# Autodesk Inventor assembly: 1000_Device
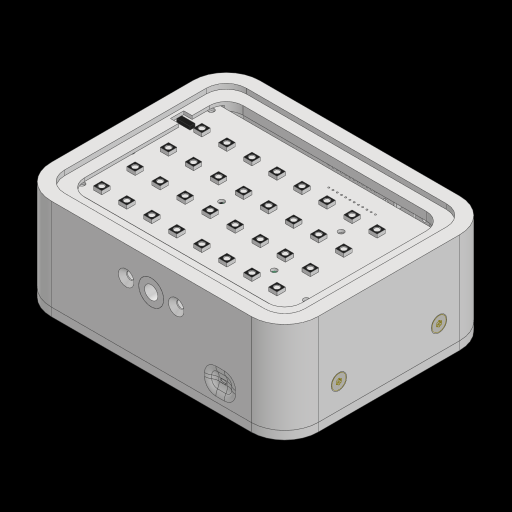
[picture p0: Inventor's stored thumbnail of the model, 512x512]
Saved by Autodesk Inventor 2024 (Build 280153000, 153)
## iProperties
Created: 2023-07-20
Part Number: 1000_Device
Document SubType Name: Assembly
Designer: Philipp
Author: Philipp
## Documents named in this file (10)
- C:\Users\phili\Documents\GitHub\PICO\20 Hardware\1000_Device.iam
- C:\Users\phili\Documents\GitHub\PICO\20 Hardware\020_Battery_4Cell.ipt
- C:\Users\phili\Documents\GitHub\PICO\20 Hardware\100_PICO_Mainboard.ipt
- C:\Users\phili\Documents\GitHub\PICO\20 Hardware\110_PICO_Daughterboard.ipt
- C:\Users\phili\Documents\GitHub\PICO\20 Hardware\SSD1306\Pantalla OLED 0.96'' 128x64.iam
- C:\Users\phili\Documents\GitHub\PICO\20 Hardware\210_Shell_External.ipt
- C:\Users\phili\Documents\GitHub\PICO\20 Hardware\220_Frame_Mainboard.ipt
- C:\Users\phili\Documents\GitHub\PICO\20 Hardware\250_CameraMount.ipt
- C:\Users\phili\Documents\GitHub\PICO\20 Hardware\241_Backplate.ipt
- C:\Users\phili\Documents\Inventor\Content Center Files\R2024\de-DE\ISO 14581_2013(E)\ISO 14581 - M4x10-4.8.ipt
## Components (12 placed, 9 different names)
1. 100_PICO_Mainboard:1 — Fluchtend:1, Fluchtend:2, Fluchtend:3, Passend:4, Fluchtend:4, Fluchtend:6, Passend:6, Fluchtend:10, Passend:10
2. 110_PICO_Daughterboard:1 — Passend:1, Passend:2, Passend:3, Passend:4, Fluchtend:4, Fluchtend:6
3. Pantalla OLED 0.96'' 128x64:1 [sub-assembly] — Passend:1, Passend:2, Passend:3
4. 210_Shell_External:1 — Passend:6, Passend:7, Passend:10, Passend:11, Passend:12, Einfügen:1, Einfügen:2, Einfügen:3, Einfügen:4, Einfügen:5
5. 220_Frame_Mainboard:1 — Passend:7, Fluchtend:10, Passend:11, Passend:12
6. 241_Backplate:1 — Passend:24
7. 020_Battery_4Cell:1 — Passend:24
8. 250_CameraMount:1 — Einfügen:1
9. Schraube ISO 14581:2013(E) M4x10-4.8:1 — Einfügen:4
10. Schraube ISO 14581:2013(E) M4x10-4.8:2 — Einfügen:3
11. Schraube ISO 14581:2013(E) M4x10-4.8:3 — Einfügen:5
12. Schraube ISO 14581:2013(E) M4x10-4.8:4 — Einfügen:2
## Relationships (26: Mate 15, Flush 6, Insert 5)
- Passend:1 [Mate]: 110_PICO_Daughterboard:1 ↔ Pantalla OLED 0.96'' 128x64:1
- Passend:2 [Mate]: 110_PICO_Daughterboard:1 ↔ Pantalla OLED 0.96'' 128x64:1
- Passend:3 [Mate]: 110_PICO_Daughterboard:1 ↔ Pantalla OLED 0.96'' 128x64:1
- Fluchtend:1 [Flush]: 100_PICO_Mainboard:1
- Fluchtend:2 [Flush]: 100_PICO_Mainboard:1
- Fluchtend:3 [Flush]: 100_PICO_Mainboard:1
- Passend:4 [Mate] (8 mm): 100_PICO_Mainboard:1 ↔ 110_PICO_Daughterboard:1
- Fluchtend:4 [Flush] (4.6 mm): 100_PICO_Mainboard:1 ↔ 110_PICO_Daughterboard:1
- Fluchtend:6 [Flush] (40.5 mm): 100_PICO_Mainboard:1 ↔ 110_PICO_Daughterboard:1
- Passend:6 [Mate] (5.5 mm): 100_PICO_Mainboard:1 ↔ 210_Shell_External:1
- Passend:7 [Mate]: 210_Shell_External:1 ↔ 220_Frame_Mainboard:1
- Fluchtend:10 [Flush]: 100_PICO_Mainboard:1 ↔ 220_Frame_Mainboard:1
- Passend:10 [Mate] (15.5 mm): 100_PICO_Mainboard:1 ↔ 210_Shell_External:1
- Passend:11 [Mate]: 210_Shell_External:1 ↔ 220_Frame_Mainboard:1
- Passend:12 [Mate]: 210_Shell_External:1 ↔ 220_Frame_Mainboard:1
- [Mate]: 210_Shell_External:1 ↔ 241_Backplate:1
- [Mate] (2 mm): 241_Backplate:1 ↔ 020_Battery_4Cell:1
- [Mate]: 210_Shell_External:1 ↔ 241_Backplate:1
- [Mate]: 210_Shell_External:1 ↔ 241_Backplate:1
- [Mate]: 241_Backplate:1 ↔ 020_Battery_4Cell:1
- Einfügen:1 [Insert] (-3 mm): 210_Shell_External:1 ↔ 250_CameraMount:1
- Passend:24 [Mate]: 241_Backplate:1 ↔ 020_Battery_4Cell:1
- Einfügen:2 [Insert]: 210_Shell_External:1 ↔ Schraube ISO 14581:2013(E) M4x10-4.8:4
- Einfügen:3 [Insert]: 210_Shell_External:1 ↔ Schraube ISO 14581:2013(E) M4x10-4.8:2
- Einfügen:4 [Insert]: 210_Shell_External:1 ↔ Schraube ISO 14581:2013(E) M4x10-4.8:1
- Einfügen:5 [Insert]: 210_Shell_External:1 ↔ Schraube ISO 14581:2013(E) M4x10-4.8:3
